# Autodesk Inventor assembly: CannonV1
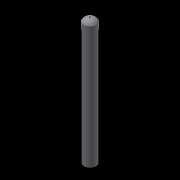
[picture p0: Inventor's stored thumbnail of the model, 180x180]
Saved by Autodesk Inventor 2019 (Build 230136000, 136)
## iProperties
Created: 2021-09-16
Part Number: CannonV1
Document SubType Name: Assembly
Designer: timmy
Author: timmy
## Documents named in this file (3)
- S:\Inventor\RoboCatz\T-Shirt\CannonV1.iam
- S:\Inventor\RoboCatz\T-Shirt\3FT-SCH40-PVC.ipt
- S:\Inventor\RoboCatz\T-Shirt\3inCAPV1.ipt
## Components (2 placed, 2 different names)
1. 3FT-SCH40-PVC:1 — Angle:1, Mate:1, Flush:1, Mate:2
2. 3inCAPV1:1 — Angle:1, Mate:1, Mate:2
## Relationships (4: Mate 2, Angle 1, Flush 1)
- Angle:1 (180 deg): 3FT-SCH40-PVC:1 ↔ 3inCAPV1:1
- Mate:1: 3FT-SCH40-PVC:1 ↔ 3inCAPV1:1
- Flush:1: 3FT-SCH40-PVC:1
- Mate:2: 3FT-SCH40-PVC:1 ↔ 3inCAPV1:1
